# Autodesk Inventor assembly: aos5
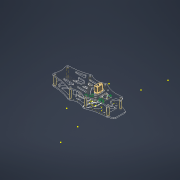
[picture p0: Inventor's stored thumbnail of the model, 180x180]
Saved by Autodesk Inventor 2022 (Build 260153000, 153)
## iProperties
Created: 2022-07-20
Part Number: aos5
Document SubType Name: Assembly
Designer: ancher
Author: ancher
## iProperties of the stored document xt60e-m.ipt
Created: 2022-05-16
Part Number: xt60e-m
Material: Generic
Document SubType Name: Modeling
Designer: ancher
Density: 1 g/cm^3
Appearance: Default
Sending System: SolidWorks 2020
Last Author: mlazor
Last Saved: 2022-05-17
Author: ancher
## Documents named in this file (12)
- E:\RC\print_3d\aos5\aos5.iam
- E:\RC\print_3d\aos5\bottom_plate.ipt
- E:\RC\print_3d\aos5\top_plate.ipt
- E:\RC\print_3d\aos5\standoff.ipt
- E:\RC\print_3d\inventor\ContentCenterFiles\en-US\ISO 7380-1\ISO 7380-1 - M3 x 6.ipt
- E:\RC\print_3d\aos5\esc.iam
- E:\RC\print_3d\inventor\ContentCenterFiles\en-US\ISO 7380-1\ISO 7380-1 - M3 x 20.ipt
- E:\RC\print_3d\inventor\ContentCenterFiles\en-US\DIN 439-2\DIN 439 - M3 x 0.5.ipt
- E:\RC\print_3d\aos5\xt60_base.ipt
- **E:\RC\print_3d\aos5\aos5.iam*LocalDocs*xAaaaqubaAaaaaaaaAaaaa5jhFc*xt60e-m.ipt
- E:\RC\print_3d\aos5\xt60h-m.ipt
- E:\RC\print_3d\aos5\xt60e-m\xt60e-m.sldprt
## Components (30 placed, 10 different names)
1. bottom_plate:1 — Mate:1, Mate:2, Mate:3, Mate:4, Mate:5, Mate:6, Mate:7, Mate:8, Mate:9, Mate:11, Mate:12, Mate:13, Mate:14, Mate:15, Mate:16, Mate:17, Mate:18, Mate:19, Mate:21, Mate:23, Mate:25, Mate:27, Mate:29, Mate:31, Mate:33, Mate:35, Mate:36, Mate:37, Insert:1, Insert:2, Insert:3, Insert:4, Mate:39, Mate:41, Mate:43, Mate:45, Flush:1
2. top_plate:1 — Mate:1, Mate:2, Mate:47
3. esc:1 [sub-assembly] — Mate:36, Mate:37, Mate:46
4. xt60_base:1 — Flush:1
5. xt60e-m:1
6. xt60h-m:1
7. DIN 439-2 - replaced by DIN EN 24035/28675 M3:1 — Mate:38, Mate:39
8. DIN 439-2 - replaced by DIN EN 24035/28675 M3:2 — Mate:40, Mate:41
9. DIN 439-2 - replaced by DIN EN 24035/28675 M3:3 — Mate:42, Mate:43
10. DIN 439-2 - replaced by DIN EN 24035/28675 M3:4 — Mate:44, Mate:45, Mate:46
11. ISO 7380-1 M3 x 20:1 — Insert:1, Mate:40
12. ISO 7380-1 M3 x 20:2 — Insert:2, Mate:42
13. ISO 7380-1 M3 x 20:3 — Insert:3, Mate:38
14. ISO 7380-1 M3 x 20:4 — Insert:4, Mate:44
15. ISO 7380-1 M3 x 6:1 — Mate:20, Mate:21
16. ISO 7380-1 M3 x 6:2 — Mate:22, Mate:23
17. ISO 7380-1 M3 x 6:3 — Mate:24, Mate:25
18. ISO 7380-1 M3 x 6:4 — Mate:26, Mate:27
19. ISO 7380-1 M3 x 6:5 — Mate:28, Mate:29
20. ISO 7380-1 M3 x 6:6 — Mate:30, Mate:31
21. ISO 7380-1 M3 x 6:7 — Mate:32, Mate:33
22. ISO 7380-1 M3 x 6:8 — Mate:34, Mate:35
23. standoff:1 — Mate:3, Mate:11, Mate:22
24. standoff:2 — Mate:4, Mate:13, Mate:24
25. standoff:3 — Mate:5, Mate:17, Mate:26
26. standoff:4 — Mate:6, Mate:19, Mate:28
27. standoff:5 — Mate:7, Mate:18, Mate:30
28. standoff:6 — Mate:8, Mate:16, Mate:32
29. standoff:7 — Mate:9, Mate:15, Mate:34, Mate:47
30. standoff:8 — Mate:12, Mate:14, Mate:20
## Relationships (51: Mate 46, Insert 4, Flush 1)
- Mate:1: bottom_plate:1 ↔ top_plate:1
- Mate:2: bottom_plate:1 ↔ top_plate:1
- Mate:3: bottom_plate:1 ↔ standoff:1
- Mate:4: bottom_plate:1 ↔ standoff:2
- Mate:5: bottom_plate:1 ↔ standoff:3
- Mate:6: bottom_plate:1 ↔ standoff:4
- Mate:7: bottom_plate:1 ↔ standoff:5
- Mate:8: bottom_plate:1 ↔ standoff:6
- Mate:9: bottom_plate:1 ↔ standoff:7
- Mate:11: bottom_plate:1 ↔ standoff:1
- Mate:12: bottom_plate:1 ↔ standoff:8
- Mate:13: bottom_plate:1 ↔ standoff:2
- Mate:14: bottom_plate:1 ↔ standoff:8
- Mate:15: bottom_plate:1 ↔ standoff:7
- Mate:16: bottom_plate:1 ↔ standoff:6
- Mate:17: bottom_plate:1 ↔ standoff:3
- Mate:18: bottom_plate:1 ↔ standoff:5
- Mate:19: bottom_plate:1 ↔ standoff:4
- Mate:20: ISO 7380-1 M3 x 6:1 ↔ standoff:8
- Mate:21: bottom_plate:1 ↔ ISO 7380-1 M3 x 6:1
- Mate:22: ISO 7380-1 M3 x 6:2 ↔ standoff:1
- Mate:23: bottom_plate:1 ↔ ISO 7380-1 M3 x 6:2
- Mate:24: ISO 7380-1 M3 x 6:3 ↔ standoff:2
- Mate:25: bottom_plate:1 ↔ ISO 7380-1 M3 x 6:3
- Mate:26: ISO 7380-1 M3 x 6:4 ↔ standoff:3
- Mate:27: bottom_plate:1 ↔ ISO 7380-1 M3 x 6:4
- Mate:28: ISO 7380-1 M3 x 6:5 ↔ standoff:4
- Mate:29: bottom_plate:1 ↔ ISO 7380-1 M3 x 6:5
- Mate:30: ISO 7380-1 M3 x 6:6 ↔ standoff:5
- Mate:31: bottom_plate:1 ↔ ISO 7380-1 M3 x 6:6
- Mate:32: ISO 7380-1 M3 x 6:7 ↔ standoff:6
- Mate:33: bottom_plate:1 ↔ ISO 7380-1 M3 x 6:7
- Mate:34: ISO 7380-1 M3 x 6:8 ↔ standoff:7
- Mate:35: bottom_plate:1 ↔ ISO 7380-1 M3 x 6:8
- Mate:36: bottom_plate:1 ↔ esc:1
- Mate:37: bottom_plate:1 ↔ esc:1
- Insert:1: bottom_plate:1 ↔ ISO 7380-1 M3 x 20:1
- Insert:2: bottom_plate:1 ↔ ISO 7380-1 M3 x 20:2
- Insert:3: bottom_plate:1 ↔ ISO 7380-1 M3 x 20:3
- Insert:4: bottom_plate:1 ↔ ISO 7380-1 M3 x 20:4
- Mate:38: DIN 439-2 - replaced by DIN EN 24035/28675 M3:1 ↔ ISO 7380-1 M3 x 20:3
- Mate:39: bottom_plate:1 ↔ DIN 439-2 - replaced by DIN EN 24035/28675 M3:1
- Mate:40: DIN 439-2 - replaced by DIN EN 24035/28675 M3:2 ↔ ISO 7380-1 M3 x 20:1
- Mate:41: bottom_plate:1 ↔ DIN 439-2 - replaced by DIN EN 24035/28675 M3:2
- Mate:42: DIN 439-2 - replaced by DIN EN 24035/28675 M3:3 ↔ ISO 7380-1 M3 x 20:2
- Mate:43: bottom_plate:1 ↔ DIN 439-2 - replaced by DIN EN 24035/28675 M3:3
- Mate:44: DIN 439-2 - replaced by DIN EN 24035/28675 M3:4 ↔ ISO 7380-1 M3 x 20:4
- Mate:45: bottom_plate:1 ↔ DIN 439-2 - replaced by DIN EN 24035/28675 M3:4
- Mate:46: esc:1 ↔ DIN 439-2 - replaced by DIN EN 24035/28675 M3:4
- Flush:1: bottom_plate:1 ↔ xt60_base:1
- Mate:47: top_plate:1 ↔ standoff:7
